# Autodesk Inventor assembly: Burner_Assembly
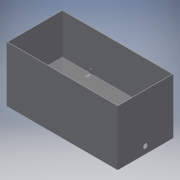
[picture p0: Inventor's stored thumbnail of the model, 180x180]
Saved by Autodesk Inventor 2017 (Build 210142000, 142)
## iProperties
Created: 2019-03-26
Part Number: Burner_Assembly
Document SubType Name: Assembly
Designer: mcgratta
Author: mcgratta
## Documents named in this file (4)
- C:\Users\mcgratta\Documents\FDS_Validation_Test_Reports\FM_Parallel_Panels\Burner_Assembly.iam
- C:\Users\mcgratta\Documents\FDS_Validation_Test_Reports\FM_Parallel_Panels\Burner.ipt
- C:\Users\mcgratta\Documents\FDS_Validation_Test_Reports\FM_Parallel_Panels\Bracket.ipt
- C:\Users\mcgratta\Documents\FDS_Validation_Test_Reports\FM_Parallel_Panels\Screen.ipt
## Components (8 placed, 3 different names)
1. Burner:1 — Mate:1, Mate:2, Mate:3, Mate:4, Flush:1, Mate:5, Flush:2, Mate:6, Mate:7, Mate:8, Flush:3, Mate:9, Flush:4, Flush:5, Mate:10, Flush:6, Mate:11, Mate:12, Mate:13, Mate:14, Flush:7
2. Bracket:1 — Mate:1, Mate:2, Mate:3
3. Bracket:2 — Mate:4, Flush:1, Mate:5
4. Bracket:3 — Flush:2, Mate:6, Mate:7
5. Bracket:4 — Mate:10, Flush:6, Mate:11
6. Bracket:5 — Flush:4, Flush:5, Mate:12
7. Bracket:6 — Mate:8, Flush:3, Mate:9
8. Screen:1 — Mate:13, Mate:14, Flush:7
## Relationships (21: Mate 14, Flush 7)
- Mate:1: Burner:1 ↔ Bracket:1
- Mate:2 (76.2 mm): Burner:1 ↔ Bracket:1
- Mate:3 (152.4 mm): Burner:1 ↔ Bracket:1
- Mate:4: Burner:1 ↔ Bracket:2
- Flush:1 (-79.375 mm): Burner:1 ↔ Bracket:2
- Mate:5 (152.4 mm): Burner:1 ↔ Bracket:2
- Flush:2 (-79.375 mm): Burner:1 ↔ Bracket:3
- Mate:6: Burner:1 ↔ Bracket:3
- Mate:7 (146.05 mm): Burner:1 ↔ Bracket:3
- Mate:8: Burner:1 ↔ Bracket:6
- Flush:3 (-79.375 mm): Burner:1 ↔ Bracket:6
- Mate:9 (152.4 mm): Burner:1 ↔ Bracket:6
- Flush:4 (-3.175 mm): Burner:1 ↔ Bracket:5
- Flush:5 (-79.375 mm): Burner:1 ↔ Bracket:5
- Mate:10: Burner:1 ↔ Bracket:4
- Flush:6 (-79.375 mm): Burner:1 ↔ Bracket:4
- Mate:11 (146.05 mm): Burner:1 ↔ Bracket:4
- Mate:12 (152.4 mm): Burner:1 ↔ Bracket:5
- Mate:13 (3.175 mm): Burner:1 ↔ Screen:1
- Mate:14 (3.175 mm): Burner:1 ↔ Screen:1
- Flush:7 (-219.075 mm): Burner:1 ↔ Screen:1
